# Autodesk Inventor assembly: Ball Shooter V5 Assembly
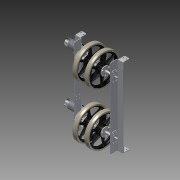
[picture p0: Inventor's stored thumbnail of the model, 180x180]
Saved by Autodesk Inventor 2014 SP1 (Build 180222100, 222)
## iProperties
Created: 2012-01-31
Part Number: Ball Shooter V5 Assembly
Document SubType Name: Assembly
Designer: Moses
Mass: 4122.24 g
Surface Area: 9874.97 cm^2
Volume: 1875.22 cm^3
Density: 2.19828 g/cm^3
Author: Moses
## Documents named in this file (9)
- C:\Users\Moses\Documents\GitHub\frc2014CAD\2012\Repackaged_Team_3061_Yr2012_Ball_Shooter\Ball Shooter V5 Assembly.iam
- C:\Users\Moses\Documents\GitHub\frc2014CAD\2012\Repackaged_Team_3061_Yr2012_Ball_Shooter\V5 Shooter Frame Channel Part 1.ipt
- C:\Users\Moses\Documents\GitHub\frc2014CAD\2012\Repackaged_Team_3061_Yr2012_Ball_Shooter\V5 Shooter Frame Channel Part 2.ipt
- C:\Users\Moses\Documents\GitHub\frc2014CAD\2012\Repackaged_Team_3061_Yr2012_Ball_Shooter\Ball Shooter Wheel Sub-Assembly V2.iam
- C:\Users\Moses\Documents\GitHub\frc2014CAD\2012\Repackaged_Team_3061_Yr2012_Ball_Shooter\V5 Shooter Frame Channel Bracket Part 3.ipt
- C:\Users\Moses\Documents\GitHub\frc2014CAD\2012\Repackaged_Team_3061_Yr2012_Ball_Shooter\Banebots RS-775 to P60 Gearbox.iam
- C:\Users\Moses\Documents\GitHub\frc2014CAD\2012\Repackaged_Team_3061_Yr2012_Ball_Shooter\fr-6-zz (1.125 OD Version).ipt
- C:\Users\Moses\Documents\GitHub\frc2014CAD\2012\Repackaged_Team_3061_Yr2012_Ball_Shooter\V5 Shooter Bearing Support Plate.ipt
- C:\Users\Moses\Documents\GitHub\frc2014CAD\2012\Repackaged_Team_3061_Yr2012_Ball_Shooter\ANSI B18.6.3 - 10-32 UNF - 0.25(14).ipt
## Components (24 placed, 8 different names)
1. Ball Shooter Wheel Sub-Assembly V2:1 [sub-assembly] — Insert:2, Rotation:2, Rotation:3
2. Ball Shooter Wheel Sub-Assembly V2:2 [sub-assembly] — Insert:1, Mate:2, Rotation:1, Rotation:3
3. Banebots RS-775 to P60 Gearbox:2 [sub-assembly] — Mate:16, Mate:19, Mate:20, Rotation:2
4. Banebots RS-775 to P60 Gearbox:1 [sub-assembly] — Mate:15, Mate:17, Mate:18, Rotation:1
5. fr-6-zz (1.125 OD Version):1 — Insert:3
6. fr-6-zz (1.125 OD Version):2 — Insert:4
7. fr-6-zz (1.125 OD Version):3 — Insert:6, Insert:7
8. fr-6-zz (1.125 OD Version):4 — Insert:5
9. V5 Shooter Bearing Support Plate:1 — Flush:2, Insert:6, Insert:7, Mate:40, Mate:41
10. V5 Shooter Bearing Support Plate:2 — Mate:21, Mate:22, Mate:23, Insert:5
11. V5 Shooter Frame Channel Bracket Part 3:4 — Mate:9, Mate:10, Mate:11
12. V5 Shooter Frame Channel Bracket Part 3:3 — Mate:12, Mate:13, Mate:14
13. V5 Shooter Frame Channel Bracket Part 3:1 — Mate:3, Mate:4, Mate:5
14. V5 Shooter Frame Channel Bracket Part 3:2 — Mate:6, Mate:7, Mate:8
15. V5 Shooter Frame Channel Part 2:1 — Mate:1, Flush:1, Mate:2, Mate:6, Mate:7, Mate:8, Mate:9, Mate:10, Mate:11, Flush:2, Mate:21, Mate:22, Mate:23, Mate:40, Mate:41
16. V5 Shooter Frame Channel Part 1:1 — Mate:1, Flush:1, Insert:1, Insert:2, Mate:3, Mate:4, Mate:5, Mate:12, Mate:13, Mate:14, Mate:15, Mate:16, Mate:17, Mate:18, Mate:19, Mate:20, Insert:3, Insert:4, Mate:25, Mate:27, Mate:29, Mate:31, Mate:33, Mate:35, Mate:37, Mate:39, Mate:26, Mate:28, Mate:30, Mate:32, Mate:34, Mate:36, Mate:38, Mate:24
17. Cross Recessed Binding Head Machine Screw - Type I - Inch No. 10 - 32 - 1/4:8 — Mate:24, Mate:25
18. Cross Recessed Binding Head Machine Screw - Type I - Inch No. 10 - 32 - 1/4:1 — Mate:26, Mate:27
19. Cross Recessed Binding Head Machine Screw - Type I - Inch No. 10 - 32 - 1/4:2 — Mate:28, Mate:29
20. Cross Recessed Binding Head Machine Screw - Type I - Inch No. 10 - 32 - 1/4:3 — Mate:30, Mate:31
21. Cross Recessed Binding Head Machine Screw - Type I - Inch No. 10 - 32 - 1/4:4 — Mate:32, Mate:33
22. Cross Recessed Binding Head Machine Screw - Type I - Inch No. 10 - 32 - 1/4:5 — Mate:34, Mate:35
23. Cross Recessed Binding Head Machine Screw - Type I - Inch No. 10 - 32 - 1/4:6 — Mate:36, Mate:37
24. Cross Recessed Binding Head Machine Screw - Type I - Inch No. 10 - 32 - 1/4:7 — Mate:38, Mate:39
## Relationships (53: Mate 41, Insert 7, RelateRotation 3, Flush 2)
- Mate:1 (228.6 mm): V5 Shooter Frame Channel Part 2:1 ↔ V5 Shooter Frame Channel Part 1:1
- Flush:1: V5 Shooter Frame Channel Part 2:1 ↔ V5 Shooter Frame Channel Part 1:1
- Insert:1 (1.6002 mm): Ball Shooter Wheel Sub-Assembly V2:2 ↔ V5 Shooter Frame Channel Part 1:1
- Insert:2 (1.6002 mm): Ball Shooter Wheel Sub-Assembly V2:1 ↔ V5 Shooter Frame Channel Part 1:1
- Mate:2: Ball Shooter Wheel Sub-Assembly V2:2 ↔ V5 Shooter Frame Channel Part 2:1
- Mate:3: V5 Shooter Frame Channel Bracket Part 3:1 ↔ V5 Shooter Frame Channel Part 1:1
- Mate:4: V5 Shooter Frame Channel Bracket Part 3:1 ↔ V5 Shooter Frame Channel Part 1:1
- Mate:5: V5 Shooter Frame Channel Bracket Part 3:1 ↔ V5 Shooter Frame Channel Part 1:1
- Mate:6: V5 Shooter Frame Channel Bracket Part 3:2 ↔ V5 Shooter Frame Channel Part 2:1
- Mate:7: V5 Shooter Frame Channel Bracket Part 3:2 ↔ V5 Shooter Frame Channel Part 2:1
- Mate:8: V5 Shooter Frame Channel Bracket Part 3:2 ↔ V5 Shooter Frame Channel Part 2:1
- Mate:9: V5 Shooter Frame Channel Bracket Part 3:4 ↔ V5 Shooter Frame Channel Part 2:1
- Mate:10: V5 Shooter Frame Channel Bracket Part 3:4 ↔ V5 Shooter Frame Channel Part 2:1
- Mate:11: V5 Shooter Frame Channel Bracket Part 3:4 ↔ V5 Shooter Frame Channel Part 2:1
- Mate:12: V5 Shooter Frame Channel Bracket Part 3:3 ↔ V5 Shooter Frame Channel Part 1:1
- Mate:13: V5 Shooter Frame Channel Bracket Part 3:3 ↔ V5 Shooter Frame Channel Part 1:1
- Mate:14: V5 Shooter Frame Channel Bracket Part 3:3 ↔ V5 Shooter Frame Channel Part 1:1
- Mate:15: Banebots RS-775 to P60 Gearbox:1 ↔ V5 Shooter Frame Channel Part 1:1
- Mate:16: Banebots RS-775 to P60 Gearbox:2 ↔ V5 Shooter Frame Channel Part 1:1
- Mate:17: Banebots RS-775 to P60 Gearbox:1 ↔ V5 Shooter Frame Channel Part 1:1
- Mate:18: Banebots RS-775 to P60 Gearbox:1 ↔ V5 Shooter Frame Channel Part 1:1
- Mate:19: Banebots RS-775 to P60 Gearbox:2 ↔ V5 Shooter Frame Channel Part 1:1
- Mate:20: Banebots RS-775 to P60 Gearbox:2 ↔ V5 Shooter Frame Channel Part 1:1
- Insert:3: fr-6-zz (1.125 OD Version):1 ↔ V5 Shooter Frame Channel Part 1:1
- Insert:4: fr-6-zz (1.125 OD Version):2 ↔ V5 Shooter Frame Channel Part 1:1
- Insert:5: fr-6-zz (1.125 OD Version):4 ↔ V5 Shooter Bearing Support Plate:2
- Flush:2: V5 Shooter Bearing Support Plate:1 ↔ V5 Shooter Frame Channel Part 2:1
- Mate:21: V5 Shooter Bearing Support Plate:2 ↔ V5 Shooter Frame Channel Part 2:1
- Mate:22: V5 Shooter Bearing Support Plate:2 ↔ V5 Shooter Frame Channel Part 2:1
- Mate:23: V5 Shooter Bearing Support Plate:2 ↔ V5 Shooter Frame Channel Part 2:1
- Insert:6: fr-6-zz (1.125 OD Version):3 ↔ V5 Shooter Bearing Support Plate:1
- Rotation:1 [RelateRotation] (0.4444 ul): Ball Shooter Wheel Sub-Assembly V2:2 ↔ Banebots RS-775 to P60 Gearbox:1
- Rotation:2 [RelateRotation] (0.4444 ul): Ball Shooter Wheel Sub-Assembly V2:1 ↔ Banebots RS-775 to P60 Gearbox:2
- Mate:25: V5 Shooter Frame Channel Part 1:1 ↔ Cross Recessed Binding Head Machine Screw - Type I - Inch No. 10 - 32 - 1/4:8
- Mate:27: V5 Shooter Frame Channel Part 1:1 ↔ Cross Recessed Binding Head Machine Screw - Type I - Inch No. 10 - 32 - 1/4:1
- Mate:29: V5 Shooter Frame Channel Part 1:1 ↔ Cross Recessed Binding Head Machine Screw - Type I - Inch No. 10 - 32 - 1/4:2
- Mate:31: V5 Shooter Frame Channel Part 1:1 ↔ Cross Recessed Binding Head Machine Screw - Type I - Inch No. 10 - 32 - 1/4:3
- Mate:33: V5 Shooter Frame Channel Part 1:1 ↔ Cross Recessed Binding Head Machine Screw - Type I - Inch No. 10 - 32 - 1/4:4
- Mate:35: V5 Shooter Frame Channel Part 1:1 ↔ Cross Recessed Binding Head Machine Screw - Type I - Inch No. 10 - 32 - 1/4:5
- Mate:37: V5 Shooter Frame Channel Part 1:1 ↔ Cross Recessed Binding Head Machine Screw - Type I - Inch No. 10 - 32 - 1/4:6
- Mate:39: V5 Shooter Frame Channel Part 1:1 ↔ Cross Recessed Binding Head Machine Screw - Type I - Inch No. 10 - 32 - 1/4:7
- Rotation:3 [RelateRotation] (1 ul): Ball Shooter Wheel Sub-Assembly V2:1 ↔ Ball Shooter Wheel Sub-Assembly V2:2
- Mate:24: V5 Shooter Frame Channel Part 1:1 ↔ Cross Recessed Binding Head Machine Screw - Type I - Inch No. 10 - 32 - 1/4:8
- Mate:26: V5 Shooter Frame Channel Part 1:1 ↔ Cross Recessed Binding Head Machine Screw - Type I - Inch No. 10 - 32 - 1/4:1
- Mate:28: V5 Shooter Frame Channel Part 1:1 ↔ Cross Recessed Binding Head Machine Screw - Type I - Inch No. 10 - 32 - 1/4:2
- Mate:30: V5 Shooter Frame Channel Part 1:1 ↔ Cross Recessed Binding Head Machine Screw - Type I - Inch No. 10 - 32 - 1/4:3
- Mate:32: V5 Shooter Frame Channel Part 1:1 ↔ Cross Recessed Binding Head Machine Screw - Type I - Inch No. 10 - 32 - 1/4:4
- Mate:34: V5 Shooter Frame Channel Part 1:1 ↔ Cross Recessed Binding Head Machine Screw - Type I - Inch No. 10 - 32 - 1/4:5
- Mate:36: V5 Shooter Frame Channel Part 1:1 ↔ Cross Recessed Binding Head Machine Screw - Type I - Inch No. 10 - 32 - 1/4:6
- Mate:38: V5 Shooter Frame Channel Part 1:1 ↔ Cross Recessed Binding Head Machine Screw - Type I - Inch No. 10 - 32 - 1/4:7
- Insert:7: fr-6-zz (1.125 OD Version):3 ↔ V5 Shooter Bearing Support Plate:1
- Mate:40: V5 Shooter Bearing Support Plate:1 ↔ V5 Shooter Frame Channel Part 2:1
- Mate:41: V5 Shooter Bearing Support Plate:1 ↔ V5 Shooter Frame Channel Part 2:1
